# Autodesk Inventor assembly: 6P 8T Sprocket, No Insert
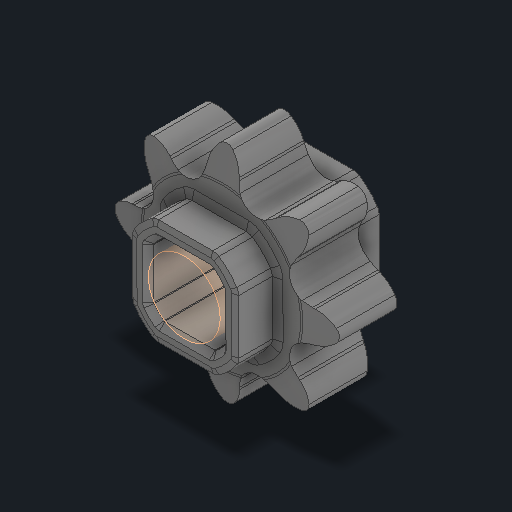
[picture p0: Inventor's stored thumbnail of the model, 512x512]
Saved by Autodesk Inventor 2025.1 (Build 291241000, 241)
## iProperties
Created: 2022-08-02
Part Number: 6P 8T Sprocket, No Insert
Document SubType Name: Assembly
Designer: avere
Author: ylu12
## Documents named in this file (2)
- C:\Users\avere\VEX\High Stakes\CAD\V3\Intake\Gearbox Right\6P 8T Sprocket, No Insert.iam
- C:\Users\avere\VEX\High Stakes\CAD\V3\Intake\Gearbox Right\6P 8T Sprocket.ipt
## Components (1 placed, 1 different names)
1. 6P 8T Sprocket:1 — Flush:3, Mate:6, Mate:5
## Relationships (3: Mate 2, Flush 1)
- Flush:3: 6P 8T Sprocket:1
- Mate:6: 6P 8T Sprocket:1
- Mate:5: 6P 8T Sprocket:1
